# Autodesk Inventor assembly: FilmLamp
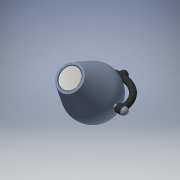
[picture p0: Inventor's stored thumbnail of the model, 180x180]
Saved by Autodesk Inventor 2018.2 (Build 222227000, 227)
## iProperties
Created: 2018-02-01
Part Number: FilmLamp
Material: Generisch
Document SubType Name: Assembly
Designer: JochenAlt
Author: JochenAlt
## Documents named in this file (5)
- D:\Projects\concretelamp\CAD\Vulcano\FilmLamp.iam
- D:\Projects\concretelamp\CAD\Vulcano\FilmLampHolder.ipt
- D:\Projects\concretelamp\CAD\Vulcano\FilmLamp.ipt
- D:\Projects\concretelamp\CAD\Bulb GU10\Bulb GU10.iam
- D:\Projects\concretelamp\CAD\Vulcano\FilmLamp-Clamp.ipt
## Components (5 placed, 4 different names)
1. FilmLampHolder:1 — Passend:1, Passend:2, Passend:4, Passend:5, Passend:6, Passend:7
2. Lamp:1 — Passend:1, Passend:2, Passend:3, Fluchtend:1
3. Bulb GU10:1 [sub-assembly] — Passend:3, Fluchtend:1
4. FilmLamp-Clamp:1 — Passend:4, Passend:7
5. FilmLamp-Clamp:2 — Passend:5, Passend:6
## Relationships (8: Mate 7, Flush 1)
- Passend:1 [Mate]: FilmLampHolder:1 ↔ Lamp:1
- Passend:2 [Mate] (7.5 mm): FilmLampHolder:1 ↔ Lamp:1
- Passend:3 [Mate]: Lamp:1 ↔ Bulb GU10:1
- Fluchtend:1 [Flush]: Lamp:1 ↔ Bulb GU10:1
- Passend:4 [Mate]: FilmLampHolder:1 ↔ FilmLamp-Clamp:1
- Passend:5 [Mate]: FilmLampHolder:1 ↔ FilmLamp-Clamp:2
- Passend:6 [Mate]: FilmLampHolder:1 ↔ FilmLamp-Clamp:2
- Passend:7 [Mate]: FilmLampHolder:1 ↔ FilmLamp-Clamp:1
